# Autodesk Inventor assembly: Spool Assembly
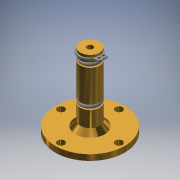
[picture p0: Inventor's stored thumbnail of the model, 180x180]
Saved by Autodesk Inventor 2019.4 (Build 234330000, 330)
## iProperties
Created: 2021-01-08
Part Number: Spool Assembly
Document SubType Name: Assembly
Designer: caleb
Author: caleb
## Documents named in this file (4)
- C:\Users\cfang\Desktop\nebraska-silicon-lab\CAD\ETL\Module Assembly\Picker Tool\Spool Assembly.iam
- C:\Users\cfang\Desktop\nebraska-silicon-lab\CAD\ETL\Module Assembly\Picker Tool\Picker Spool.ipt
- C:\Users\cfang\Desktop\nebraska-silicon-lab\CAD\ETL\Module Assembly\Picker Tool\91590A115_STAINLESS STEEL EXTERNAL RETAINING RING.ipt
- C:\Users\cfang\Desktop\nebraska-silicon-lab\CAD\ETL\Module Assembly\Picker Tool\9452K160_OIL-RESISTANT BUNA-N MULTIPURPOSE O-RING.ipt
## Components (5 placed, 3 different names)
1. Picker Spool:1 — Insert:1, Rigid:1, Rigid:2, Rigid:3
2. 91590A115_STAINLESS STEEL EXTERNAL RETAINING RING:1 — Insert:1
3. 9452K160_OIL-RESISTANT BUNA-N MULTIPURPOSE O-RING:1 — Rigid:1
4. 9452K160_OIL-RESISTANT BUNA-N MULTIPURPOSE O-RING:2 — Rigid:2
5. 9452K160_OIL-RESISTANT BUNA-N MULTIPURPOSE O-RING:3 — Rigid:3
## Relationships (4: WeldJoint 3, Insert 1)
- Insert:1: Picker Spool:1 ↔ 91590A115_STAINLESS STEEL EXTERNAL RETAINING RING:1
- Rigid:1 [WeldJoint]: Picker Spool:1 ↔ 9452K160_OIL-RESISTANT BUNA-N MULTIPURPOSE O-RING:1
- Rigid:2 [WeldJoint]: Picker Spool:1 ↔ 9452K160_OIL-RESISTANT BUNA-N MULTIPURPOSE O-RING:2
- Rigid:3 [WeldJoint] (-0.508 mm): Picker Spool:1 ↔ 9452K160_OIL-RESISTANT BUNA-N MULTIPURPOSE O-RING:3
